# Autodesk Inventor assembly: bay_assembly
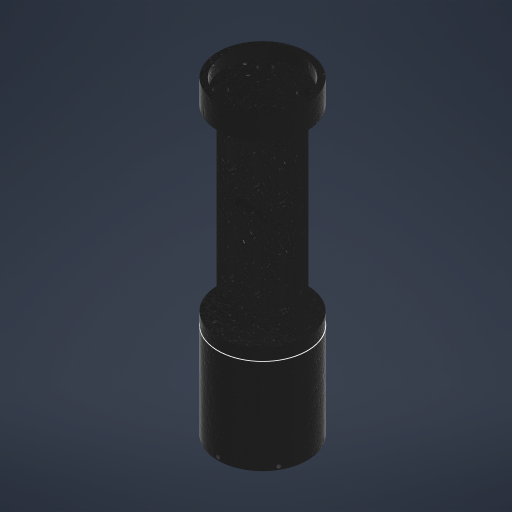
[picture p0: Inventor's stored thumbnail of the model, 512x512]
Saved by Autodesk Inventor 2023 (Build 270158000, 158)
## iProperties
Created: 2022-11-18
Part Number: bay_assembly
Document SubType Name: Assembly
Designer: washington
Author: washington
## Documents named in this file (5)
- C:\Users\washi\Desktop\NAKUJA\N2AvionicsBayDesign\bay_assembly.iam
- C:\Users\washi\Desktop\NAKUJA\N2AvionicsBayDesign\battery_holder_75mm\battery_holder_75mm.ipt
- C:\Users\washi\Desktop\NAKUJA\N2AvionicsBayDesign\bay_bottom_75mm\bay_bottom_75mm.ipt
- C:\Users\washi\Desktop\NAKUJA\N2AvionicsBayDesign\bay_mid_75mm\bay_mid_75mm.ipt
- C:\Users\washi\Desktop\NAKUJA\N2AvionicsBayDesign\bay_top_75mm\bay_top_75mm.ipt
## Components (4 placed, 4 different names)
1. battery_holder_75mm:1 — Mate:1, Mate:2, Rotational:1
2. bay_bottom_75mm:1 — Mate:1, Mate:2, Rotational:1, Mate:3, Mate:4, Mate:5
3. bay_mid_75mm:1 — Mate:3, Mate:4, Mate:5, Mate:6, Mate:7, Mate:8
4. bay_top_75mm:1 — Mate:6, Mate:7, Mate:8
## Relationships (9: Mate 8, RevoluteJoint 1)
- Mate:1: battery_holder_75mm:1 ↔ bay_bottom_75mm:1
- Mate:2: battery_holder_75mm:1 ↔ bay_bottom_75mm:1
- Rotational:1 [RevoluteJoint]: battery_holder_75mm:1 ↔ bay_bottom_75mm:1
- Mate:3: bay_bottom_75mm:1 ↔ bay_mid_75mm:1
- Mate:4: bay_bottom_75mm:1 ↔ bay_mid_75mm:1
- Mate:5: bay_bottom_75mm:1 ↔ bay_mid_75mm:1
- Mate:6: bay_mid_75mm:1 ↔ bay_top_75mm:1
- Mate:7: bay_mid_75mm:1 ↔ bay_top_75mm:1
- Mate:8: bay_mid_75mm:1 ↔ bay_top_75mm:1
